# Autodesk Inventor assembly: 8in Cyl
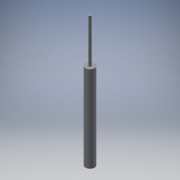
[picture p0: Inventor's stored thumbnail of the model, 180x180]
Saved by Autodesk Inventor 2018 (Build 220112000, 112)
## iProperties
Created: 2018-01-26
Part Number: 8in Cyl
Document SubType Name: Assembly
Designer: Apple
Author: Apple
## Documents named in this file (3)
- C:\Users\Apple\Documents\Inventor\2018 PowerUp\Cube Intake\8in Cyl.iam
- C:\Users\Apple\Documents\Inventor\2018 PowerUp\Cube Intake\Cylinder.ipt
- C:\Users\Apple\Documents\Inventor\2018 PowerUp\Cube Intake\Cyl_Rod.ipt
## Components (2 placed, 2 different names)
1. Cylinder:1 — Cylindrical:1
2. Cyl_Rod:1 — Flush:1, Cylindrical:1
## Relationships (2: Flush 1, CylindricalJoint 1)
- Flush:1: Cyl_Rod:1
- Cylindrical:1: Cylinder:1 ↔ Cyl_Rod:1
